# Autodesk Inventor assembly: Thorax
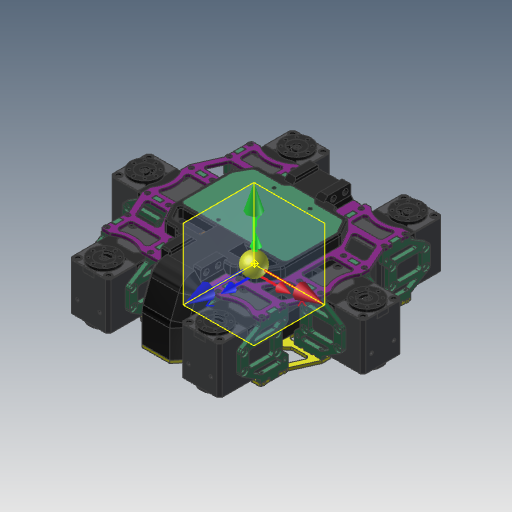
[picture p0: Inventor's stored thumbnail of the model, 512x512]
Saved by Autodesk Inventor 2019.4 (Build 234330000, 330)
## iProperties
Created: 2018-08-06
Part Number: Thorax
Material: 一般
Document SubType Name: Assembly
Designer: student
Mass: 676.028 g
Surface Area: 2162.31 cm^2
Volume: 512.52 cm^3
Density: 1.31903 g/cm^3
Author: student
## Documents named in this file (11)
- C:\Workspace\HaptHexa\Hardware\Inventor\Thorax\_Thorax.iam
- C:\Workspace\HaptHexa\Hardware\Inventor\Thorax\yaw_unit\yaw_unit.iam
- C:\Workspace\HaptHexa\Hardware\Inventor\Thorax\kypom_3s_2500.ipt
- C:\Workspace\HaptHexa\Hardware\Inventor\Thorax\U2D2.ipt
- C:\Workspace\HaptHexa\Hardware\Inventor\Thorax\body_bottom.ipt
- C:\Workspace\HaptHexa\Hardware\Inventor\Thorax\body_top.ipt
- C:\Workspace\HaptHexa\Hardware\Inventor\Thorax\battery_cover_v2.ipt
- C:\Workspace\HaptHexa\Hardware\Inventor\Thorax\battery_holder_back.ipt
- C:\Workspace\HaptHexa\Hardware\Inventor\Thorax\battery_lib_assy.iam
- C:\Workspace\HaptHexa\Hardware\Inventor\Thorax\body_top_mir.ipt
- C:\Workspace\HaptHexa\Hardware\Inventor\Thorax\main_pcb.ipt
## Components (15 placed, 10 different names)
1. battery_cover_v2:1 — フラッシュ:1, フラッシュ:2, フラッシュ:3, メイト:46, メイト:47, メイト:48, メイト:49, メイト:50
2. kypom_3s_2500:1
3. U2D2:1 — メイト:45, メイト:46, メイト:48
4. body_bottom:1 — メイト:4, メイト:5, メイト:17, メイト:18, メイト:23, メイト:24, メイト:26, メイト:27, フラッシュ:51, フラッシュ:52, フラッシュ:53, メイト:49, メイト:52, メイト:53, メイト:54, メイト:55, メイト:56, メイト:57, メイト:58, メイト:59, メイト:60
5. battery_holder_back:1 — メイト:20, フラッシュ:5, メイト:34, メイト:35, メイト:50, メイト:51
6. battery_lib_assy:1 [sub-assembly] — メイト:34, メイト:35, メイト:51
7. body_top:1 — メイト:42, メイト:43, フラッシュ:6
8. body_top_mir:1 — メイト:61, メイト:62, メイト:63
9. main_pcb:1 — メイト:47, フラッシュ:49, フラッシュ:50
10. yaw_unit:4 [sub-assembly] — メイト:52, メイト:53, メイト:54, メイト:61, メイト:62, メイト:63
11. yaw_unit:5 [sub-assembly] — メイト:55, メイト:56, メイト:57
12. yaw_unit:6 [sub-assembly] — メイト:58, メイト:59, メイト:60
13. yaw_unit:1 [sub-assembly] — メイト:26, メイト:27, フラッシュ:51
14. yaw_unit:2 [sub-assembly] — メイト:23, メイト:24, メイト:42, メイト:43, フラッシュ:6, フラッシュ:52
15. yaw_unit:3 [sub-assembly] — メイト:17, メイト:18, メイト:45, フラッシュ:53
## Relationships (42: Mate 32, Flush 10)
- メイト:4 [Mate]: body_bottom:1
- メイト:5 [Mate]: body_bottom:1
- フラッシュ:1 [Flush]: battery_cover_v2:1
- フラッシュ:2 [Flush] (-13 mm): battery_cover_v2:1
- フラッシュ:3 [Flush]: battery_cover_v2:1
- メイト:17 [Mate]: body_bottom:1 ↔ yaw_unit:3
- メイト:18 [Mate]: body_bottom:1 ↔ yaw_unit:3
- メイト:20 [Mate]: battery_holder_back:1
- フラッシュ:5 [Flush]: battery_holder_back:1
- メイト:23 [Mate]: body_bottom:1 ↔ yaw_unit:2
- メイト:24 [Mate]: body_bottom:1 ↔ yaw_unit:2
- メイト:26 [Mate]: body_bottom:1 ↔ yaw_unit:1
- メイト:27 [Mate]: body_bottom:1 ↔ yaw_unit:1
- メイト:34 [Mate]: battery_holder_back:1 ↔ battery_lib_assy:1
- メイト:35 [Mate]: battery_holder_back:1 ↔ battery_lib_assy:1
- メイト:42 [Mate]: body_top:1 ↔ yaw_unit:2
- メイト:43 [Mate]: body_top:1 ↔ yaw_unit:2
- フラッシュ:6 [Flush]: body_top:1 ↔ yaw_unit:2
- メイト:45 [Mate] (2 mm): U2D2:1 ↔ yaw_unit:3
- メイト:46 [Mate] (3 mm): battery_cover_v2:1 ↔ U2D2:1
- メイト:47 [Mate]: battery_cover_v2:1 ↔ main_pcb:1
- フラッシュ:49 [Flush]: main_pcb:1
- フラッシュ:50 [Flush]: main_pcb:1
- メイト:48 [Mate]: battery_cover_v2:1 ↔ U2D2:1
- フラッシュ:51 [Flush]: body_bottom:1 ↔ yaw_unit:1
- フラッシュ:52 [Flush]: body_bottom:1 ↔ yaw_unit:2
- フラッシュ:53 [Flush]: body_bottom:1 ↔ yaw_unit:3
- メイト:49 [Mate]: battery_cover_v2:1 ↔ body_bottom:1
- メイト:50 [Mate]: battery_cover_v2:1 ↔ battery_holder_back:1
- メイト:51 [Mate]: battery_holder_back:1 ↔ battery_lib_assy:1
- メイト:52 [Mate]: body_bottom:1 ↔ yaw_unit:4
- メイト:53 [Mate]: body_bottom:1 ↔ yaw_unit:4
- メイト:54 [Mate]: body_bottom:1 ↔ yaw_unit:4
- メイト:55 [Mate]: body_bottom:1 ↔ yaw_unit:5
- メイト:56 [Mate]: body_bottom:1 ↔ yaw_unit:5
- メイト:57 [Mate]: body_bottom:1 ↔ yaw_unit:5
- メイト:58 [Mate]: body_bottom:1 ↔ yaw_unit:6
- メイト:59 [Mate]: body_bottom:1 ↔ yaw_unit:6
- メイト:60 [Mate]: body_bottom:1 ↔ yaw_unit:6
- メイト:61 [Mate]: body_top_mir:1 ↔ yaw_unit:4
- メイト:62 [Mate]: body_top_mir:1 ↔ yaw_unit:4
- メイト:63 [Mate]: body_top_mir:1 ↔ yaw_unit:4
